# Autodesk Inventor assembly: rig_v2
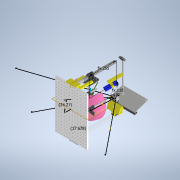
[picture p0: Inventor's stored thumbnail of the model, 180x180]
Saved by Autodesk Inventor 2022 (Build 260153000, 153)
## iProperties
Created: 2021-02-02
Part Number: rig_v2
Document SubType Name: Assembly
Designer: dsdan
Author: dsdan
## Documents named in this file (33)
- E:\OneDrive - Imperial College London\DragonVision_DanielKo\Instrumentation\Ephys_rig_2021\rig_v2.iam
- E:\OneDrive - Imperial College London\DragonVision_DanielKo\Instrumentation\Ephys_rig_2021\Imported Components\MB3045U_M-Solidworks\MB3045U_M-Solidworks.ipt
- E:\OneDrive - Imperial College London\DragonVision_DanielKo\Instrumentation\Ephys_rig_2021\Imported Components\TR150_M-Solidworks\TR150_M-Solidworks.ipt
- E:\OneDrive - Imperial College London\DragonVision_DanielKo\Instrumentation\Ephys_rig_2021\Imported Components\XT34-500-Solidworks\XT34-500-Solidworks.ipt
- E:\OneDrive - Imperial College London\DragonVision_DanielKo\Instrumentation\Ephys_rig_2021\Imported Components\XT34HP_M-Solidworks\XT34HP_M-Solidworks.ipt
- E:\OneDrive - Imperial College London\DragonVision_DanielKo\Instrumentation\Ephys_rig_2021\Imported Components\UPH50_M-Solidworks\UPH50_M-Solidworks.ipt
- E:\OneDrive - Imperial College London\DragonVision_DanielKo\Instrumentation\Ephys_rig_2021\Imported Components\BA2R_M-Solidworks\BA2R_M-Solidworks.ipt
- E:\OneDrive - Imperial College London\DragonVision_DanielKo\Instrumentation\Ephys_rig_2021\Dome\dome_assembly.iam
- E:\OneDrive - Imperial College London\DragonVision_DanielKo\Instrumentation\Ephys_rig_2021\Imported Components\TR100_M-Solidworks.ipt
- E:\OneDrive - Imperial College London\DragonVision_DanielKo\Instrumentation\Ephys_rig_2021\Imported Components\RA90_M-Solidworks.ipt
- E:\OneDrive - Imperial College London\DragonVision_DanielKo\Instrumentation\Ephys_rig_2021\Projector_swing v2\swing_assembly.iam
- E:\OneDrive - Imperial College London\DragonVision_DanielKo\Instrumentation\Ephys_rig_2021\RP01_M-Solidworks.ipt
- E:\OneDrive - Imperial College London\DragonVision_DanielKo\Instrumentation\Ephys_rig_2021\dragonfly_head.ipt
- E:\OneDrive - Imperial College London\DragonVision_DanielKo\Instrumentation\Ephys_rig_2021\Imported Components\XE25L225_M-Solidworks.ipt
- E:\OneDrive - Imperial College London\DragonVision_DanielKo\Instrumentation\Ephys_rig_2021\Holder\head_adjustable_v4.ipt
- E:\OneDrive - Imperial College London\DragonVision_DanielKo\Instrumentation\Ephys_rig_2021\electrode.ipt
- E:\OneDrive - Imperial College London\DragonVision_DanielKo\Instrumentation\Ephys_rig_2021\Dinolite.ipt
- E:\OneDrive - Imperial College London\DragonVision_DanielKo\Instrumentation\Ephys_rig_2021\endoscope.ipt
- E:\OneDrive - Imperial College London\DragonVision_DanielKo\Instrumentation\Ephys_rig_2021\projector.ipt
- E:\OneDrive - Imperial College London\DragonVision_DanielKo\Instrumentation\Ephys_rig_2021\dinolite_holder.iam
- E:\OneDrive - Imperial College London\DragonVision_DanielKo\Instrumentation\Ephys_rig_2021\Imported Components\RS100P4_M-Solidworks\RS100P4_M-Solidworks.ipt
- E:\OneDrive - Imperial College London\DragonVision_DanielKo\Instrumentation\Ephys_rig_2021\Imported Components\RS4P_M-Solidworks\RS4P_M-Solidworks.ipt
- E:\OneDrive - Imperial College London\DragonVision_DanielKo\Instrumentation\Ephys_rig_2021\Imported Components\CF125C_M-Solidworks\CF125C_M-Solidworks.ipt
- E:\OneDrive - Imperial College London\DragonVision_DanielKo\Instrumentation\Ephys_rig_2021\C1045_M-Solidworks.ipt
- E:\OneDrive - Imperial College London\DragonVision_DanielKo\Instrumentation\Ephys_rig_2021\pillar_placer.ipt
- E:\OneDrive - Imperial College London\DragonVision_DanielKo\Instrumentation\Ephys_rig_2021\head_lock_2.ipt
- E:\OneDrive - Imperial College London\DragonVision_DanielKo\Instrumentation\Ephys_rig_2021\domePlace.ipt
- E:\OneDrive - Imperial College London\DragonVision_DanielKo\Instrumentation\Ephys_rig_2021\domePlaceSingle.ipt
- E:\OneDrive - Imperial College London\DragonVision_DanielKo\Instrumentation\Ephys_rig_2021\angle_pointer.ipt
- E:\OneDrive - Imperial College London\DragonVision_DanielKo\Instrumentation\Ephys_rig_2021\stringHold.ipt
- E:\OneDrive - Imperial College London\DragonVision_DanielKo\Instrumentation\Ephys_rig_2021\projectorPlace.ipt
- E:\OneDrive - Imperial College London\DragonVision_DanielKo\Instrumentation\Ephys_rig_2021\rotator_squarer.ipt
- E:\OneDrive - Imperial College London\DragonVision_DanielKo\Instrumentation\Ephys_rig_2021\axis_module_v2.iam
## Components (46 placed, 32 different names)
1. MB3045U_M-Solidworks:1 — Flush:1, Mate:1, Mate:10, Mate:36, Angle:2, Tangent:24, Angle:3, Angle:4, Angle:6, Mate:169, Tangent:28, Mate:208, Mate:210, Flush:195, Mate:235, Mate:255, Mate:278, Mate:283, Mate:284, Mate:285, Mate:286, Mate:287, Mate:303, Mate:306, Angle:10, Angle:15, Flush:198, Mate:323, Angle:16, Mate:344, Mate:356, Mate:357, Mate:359
2. TR150_M-Solidworks:1 — Mate:34, Mate:40, Mate:39
3. TR150_M-Solidworks:2 — Mate:41, Mate:43, Mate:207
4. TR150_M-Solidworks:3 — Mate:42, Mate:44, Mate:290
5. UPH50_M-Solidworks:6 — Mate:207, Mate:208, Mate:304
6. UPH50_M-Solidworks:2 — Mate:34, Mate:36, Mate:305
7. UPH50_M-Solidworks:7 — Mate:210, Mate:302
8. dome_assembly:1 [sub-assembly] — Mate:40, Mate:39, Mate:41, Mate:42, Mate:43, Mate:44, Angle:2, Flush:195, Mate:245, Mate:246, Mate:289, Mate:324, Mate:348, Mate:352
9. BA2R_M-Solidworks:1 — Mate:9, Mate:10, Tangent:24, Angle:3, Mate:85
10. XT34-500-Solidworks:1 — Mate:9, Mate:16, Mate:17, Angle:4, Mate:85
11. XT34HP_M-Solidworks:1 — Mate:16, Mate:17, Mate:115, Mate:116, Mate:117
12. swing_assembly:1 [sub-assembly] — Mate:115, Mate:116, Mate:117, Mate:201, Flush:185, Flush:186
13. projector:1 — Mate:347, Flush:349, Mate:348, Mate:349, Mate:350, Mate:351, Mate:352, Mate:353
14. axis_module_v2:1 [sub-assembly] — Mate:343, Mate:345, Mate:346, Mate:354, Mate:355, Mate:356
15. UPH50_M-Solidworks:5 — Mate:169, Mate:172, Tangent:28, Mate:255
16. TR100_M-Solidworks:5 — Mate:172
17. head_adjustable_v4:1 — Mate:343, Mate:354, Mate:374, Mate:375
18. electrode:1 — Mate:185, Mate:190
19. dragonfly_head:1 — Mate:185, Mate:190, Mate:236, Mate:247, Mate:298, Mate:327, Mate:355
20. dragonfly_head:3 — Mate:219, Mate:220, Mate:236
21. dragonfly_head:5 — Mate:245, Mate:246, Mate:247
22. Dinolite:1 — Mate:216, Flush:192, Mate:219, Mate:220
23. endoscope:1 — Mate:327
24. XE25L225_M-Solidworks:2 — Mate:201, Flush:185, Flush:186, Mate:347, Flush:349
25. dinolite_holder:1 [sub-assembly] — Mate:216, Flush:192
26. RA90_M-Solidworks:3 — Mate:364, Mate:365, Mate:366, Flush:350
27. RP01_M-Solidworks:1 — Angle:6, Mate:273, Mate:274, Angle:8, Mate:345, Mate:346
28. RS100P4_M-Solidworks:1 — Mate:275, Mate:276, Mate:277, Mate:363
29. RS4P_M-Solidworks:1 — Mate:276, Mate:277, Mate:278, Mate:279, Mate:285, Mate:288
30. CF125C_M-Solidworks:1 — Mate:279, Mate:283, Mate:284
31. C1045_M-Solidworks:1 — Mate:273, Mate:274, Angle:8, Mate:275, Mate:317, Mate:318, Angle:14, Mate:322, Mate:358
32. pillar_placer:1 — Mate:286, Mate:287, Mate:288
33. head_lock_2:1 — Mate:374, Mate:375, Mate:376
34. TR100_M-Solidworks:6 — Mate:289, Mate:290, Mate:376
35. domePlaceSingle:1 — Mate:305, Mate:306, Angle:10
36. domePlace:1 — Mate:302, Mate:303, Mate:304
37. angle_pointer:1 — Mate:317, Mate:318, Angle:14
38. stringHold:1 — Mate:349, Mate:350, Mate:351
39. projectorPlace:1 — Angle:15, Mate:344
40. rotator_squarer:1 — Flush:198, Mate:322, Mate:323
41. rotator_squarer:2 — Mate:357, Mate:358, Mate:359
42. RS100P4_M-Solidworks:2 — Mate:363, Mate:364, Mate:371, Mate:372
43. TR100_M-Solidworks:7 — Mate:366, Flush:350, Mate:367, Mate:368
44. TR100_M-Solidworks:8 — Mate:367, Mate:368, Mate:369, Mate:370
45. TR100_M-Solidworks:9 — Mate:369, Mate:370
46. RS100P4_M-Solidworks:3 — Mate:371, Mate:372, Mate:365
## Relationships (110: Mate 91, Angle 9, Flush 8, Tangent 2)
- Flush:1: MB3045U_M-Solidworks:1
- Mate:1: MB3045U_M-Solidworks:1
- Mate:9: BA2R_M-Solidworks:1 ↔ XT34-500-Solidworks:1
- Mate:10: MB3045U_M-Solidworks:1 ↔ BA2R_M-Solidworks:1
- Mate:16: XT34-500-Solidworks:1 ↔ XT34HP_M-Solidworks:1
- Mate:17: XT34-500-Solidworks:1 ↔ XT34HP_M-Solidworks:1
- Mate:34: TR150_M-Solidworks:1 ↔ UPH50_M-Solidworks:2
- Mate:36: MB3045U_M-Solidworks:1 ↔ UPH50_M-Solidworks:2
- Mate:40: TR150_M-Solidworks:1 ↔ dome_assembly:1
- Mate:39: TR150_M-Solidworks:1 ↔ dome_assembly:1
- Mate:41: TR150_M-Solidworks:2 ↔ dome_assembly:1
- Mate:42: TR150_M-Solidworks:3 ↔ dome_assembly:1
- Mate:43: TR150_M-Solidworks:2 ↔ dome_assembly:1
- Mate:44: TR150_M-Solidworks:3 ↔ dome_assembly:1
- Angle:2 (180 deg): MB3045U_M-Solidworks:1 ↔ dome_assembly:1
- Tangent:24: MB3045U_M-Solidworks:1 ↔ BA2R_M-Solidworks:1
- Angle:3 (0 deg): MB3045U_M-Solidworks:1 ↔ BA2R_M-Solidworks:1
- Angle:4 (0 deg): MB3045U_M-Solidworks:1 ↔ XT34-500-Solidworks:1
- Mate:85: BA2R_M-Solidworks:1 ↔ XT34-500-Solidworks:1
- Mate:115: XT34HP_M-Solidworks:1 ↔ swing_assembly:1
- Mate:116: XT34HP_M-Solidworks:1 ↔ swing_assembly:1
- Mate:117: XT34HP_M-Solidworks:1 ↔ swing_assembly:1
- Angle:6 (180 deg): MB3045U_M-Solidworks:1 ↔ RP01_M-Solidworks:1
- Mate:169: MB3045U_M-Solidworks:1 ↔ UPH50_M-Solidworks:5
- Mate:172: UPH50_M-Solidworks:5 ↔ TR100_M-Solidworks:5
- Tangent:28: MB3045U_M-Solidworks:1 ↔ UPH50_M-Solidworks:5
- Mate:185: electrode:1 ↔ dragonfly_head:1
- Mate:190 (25 mm): electrode:1 ↔ dragonfly_head:1
- Mate:201: swing_assembly:1 ↔ XE25L225_M-Solidworks:2
- Flush:185: swing_assembly:1 ↔ XE25L225_M-Solidworks:2
- Flush:186 (-10 mm): swing_assembly:1 ↔ XE25L225_M-Solidworks:2
- Mate:207: TR150_M-Solidworks:2 ↔ UPH50_M-Solidworks:6
- Mate:208: MB3045U_M-Solidworks:1 ↔ UPH50_M-Solidworks:6
- Mate:210: MB3045U_M-Solidworks:1 ↔ UPH50_M-Solidworks:7
- Mate:216: Dinolite:1 ↔ dinolite_holder:1
- Flush:192 (-50 mm): Dinolite:1 ↔ dinolite_holder:1
- Mate:219: dragonfly_head:3 ↔ Dinolite:1
- Mate:220 (110 mm): dragonfly_head:3 ↔ Dinolite:1
- Flush:195 (160 mm): MB3045U_M-Solidworks:1 ↔ dome_assembly:1
- Mate:235: MB3045U_M-Solidworks:1
- Mate:236: dragonfly_head:1 ↔ dragonfly_head:3
- Mate:245: dome_assembly:1 ↔ dragonfly_head:5
- Mate:246: dome_assembly:1 ↔ dragonfly_head:5
- Mate:247: dragonfly_head:1 ↔ dragonfly_head:5
- Mate:255: MB3045U_M-Solidworks:1 ↔ UPH50_M-Solidworks:5
- Mate:273: RP01_M-Solidworks:1 ↔ C1045_M-Solidworks:1
- Mate:274: RP01_M-Solidworks:1 ↔ C1045_M-Solidworks:1
- Angle:8 (0 deg): RP01_M-Solidworks:1 ↔ C1045_M-Solidworks:1
- Mate:275: RS100P4_M-Solidworks:1 ↔ C1045_M-Solidworks:1
- Mate:276: RS100P4_M-Solidworks:1 ↔ RS4P_M-Solidworks:1
- Mate:277: RS100P4_M-Solidworks:1 ↔ RS4P_M-Solidworks:1
- Mate:278: MB3045U_M-Solidworks:1 ↔ RS4P_M-Solidworks:1
- Mate:279: RS4P_M-Solidworks:1 ↔ CF125C_M-Solidworks:1
- Mate:283: MB3045U_M-Solidworks:1 ↔ CF125C_M-Solidworks:1
- Mate:284: MB3045U_M-Solidworks:1 ↔ CF125C_M-Solidworks:1
- Mate:285 (-15.875 mm): MB3045U_M-Solidworks:1 ↔ RS4P_M-Solidworks:1
- Mate:286: MB3045U_M-Solidworks:1 ↔ pillar_placer:1
- Mate:287: MB3045U_M-Solidworks:1 ↔ pillar_placer:1
- Mate:288: RS4P_M-Solidworks:1 ↔ pillar_placer:1
- Mate:289: dome_assembly:1 ↔ TR100_M-Solidworks:6
- Mate:290: TR150_M-Solidworks:3 ↔ TR100_M-Solidworks:6
- Mate:298: dragonfly_head:1
- Mate:302: UPH50_M-Solidworks:7 ↔ domePlace:1
- Mate:303: MB3045U_M-Solidworks:1 ↔ domePlace:1
- Mate:304: UPH50_M-Solidworks:6 ↔ domePlace:1
- Mate:305: UPH50_M-Solidworks:2 ↔ domePlaceSingle:1
- Mate:306: MB3045U_M-Solidworks:1 ↔ domePlaceSingle:1
- Angle:10 (0 deg): MB3045U_M-Solidworks:1 ↔ domePlaceSingle:1
- Mate:317: C1045_M-Solidworks:1 ↔ angle_pointer:1
- Mate:318: C1045_M-Solidworks:1 ↔ angle_pointer:1
- Angle:14 (0 deg): C1045_M-Solidworks:1 ↔ angle_pointer:1
- Angle:15 (0 deg): MB3045U_M-Solidworks:1 ↔ projectorPlace:1
- Flush:198: MB3045U_M-Solidworks:1 ↔ rotator_squarer:1
- Mate:322: C1045_M-Solidworks:1 ↔ rotator_squarer:1
- Mate:323: MB3045U_M-Solidworks:1 ↔ rotator_squarer:1
- Mate:324: dome_assembly:1
- Angle:16 (0 deg): MB3045U_M-Solidworks:1
- Mate:327: dragonfly_head:1 ↔ endoscope:1
- Mate:343: axis_module_v2:1 ↔ head_adjustable_v4:1
- Mate:344: MB3045U_M-Solidworks:1 ↔ projectorPlace:1
- Mate:345: axis_module_v2:1 ↔ RP01_M-Solidworks:1
- Mate:346: axis_module_v2:1 ↔ RP01_M-Solidworks:1
- Mate:347 (6 mm): projector:1 ↔ XE25L225_M-Solidworks:2
- Flush:349: projector:1 ↔ XE25L225_M-Solidworks:2
- Mate:348: dome_assembly:1 ↔ projector:1
- Mate:349: projector:1 ↔ stringHold:1
- Mate:350: projector:1 ↔ stringHold:1
- Mate:351: projector:1 ↔ stringHold:1
- Mate:352 (255 mm): dome_assembly:1 ↔ projector:1
- Mate:353 (-115 mm): projector:1
- Mate:354: axis_module_v2:1 ↔ head_adjustable_v4:1
- Mate:355 (5 mm): axis_module_v2:1 ↔ dragonfly_head:1
- Mate:356 (158 mm): MB3045U_M-Solidworks:1 ↔ axis_module_v2:1
- Mate:357: MB3045U_M-Solidworks:1 ↔ rotator_squarer:2
- Mate:358: C1045_M-Solidworks:1 ↔ rotator_squarer:2
- Mate:359: MB3045U_M-Solidworks:1 ↔ rotator_squarer:2
- Mate:363: RS100P4_M-Solidworks:1 ↔ RS100P4_M-Solidworks:2
- Mate:364: RA90_M-Solidworks:3 ↔ RS100P4_M-Solidworks:2
- Mate:365 (50 mm): RA90_M-Solidworks:3 ↔ RS100P4_M-Solidworks:3
- Mate:366: RA90_M-Solidworks:3 ↔ TR100_M-Solidworks:7
- Flush:350: RA90_M-Solidworks:3 ↔ TR100_M-Solidworks:7
- Mate:367: TR100_M-Solidworks:7 ↔ TR100_M-Solidworks:8
- Mate:368: TR100_M-Solidworks:7 ↔ TR100_M-Solidworks:8
- Mate:369: TR100_M-Solidworks:8 ↔ TR100_M-Solidworks:9
- Mate:370: TR100_M-Solidworks:8 ↔ TR100_M-Solidworks:9
- Mate:371: RS100P4_M-Solidworks:2 ↔ RS100P4_M-Solidworks:3
- Mate:372: RS100P4_M-Solidworks:2 ↔ RS100P4_M-Solidworks:3
- Mate:374: head_adjustable_v4:1 ↔ head_lock_2:1
- Mate:375: head_adjustable_v4:1 ↔ head_lock_2:1
- Mate:376: head_lock_2:1 ↔ TR100_M-Solidworks:6
## Named parameters: offsetY = 115 mm, heightZ = 255 mm
